# Autodesk Inventor assembly: Cup_Dispenser
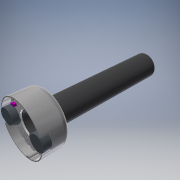
[picture p0: Inventor's stored thumbnail of the model, 180x180]
Saved by Autodesk Inventor 2016 (Build 200138000, 138)
## iProperties
Created: 2015-07-19
Part Number: Cup_Dispenser
Document SubType Name: Assembly
Designer: bastli
Author: bastli
## Documents named in this file (9)
- C:\Users\3DPrinterUser\Documents\GitHub\BarBot\Conception\Mechanical\Cup_Dispenser_3\Cup_Dispenser.iam
- C:\Users\3DPrinterUser\Documents\GitHub\BarBot\Conception\Mechanical\Cup_Dispenser_3\Fixture.ipt
- C:\Users\3DPrinterUser\Documents\GitHub\BarBot\Conception\Mechanical\Cup_Dispenser_3\Transmission.ipt
- C:\Users\3DPrinterUser\Documents\GitHub\BarBot\Conception\Mechanical\Cup_Dispenser\Cup_Dispenser_Pipe.ipt
- C:\Users\3DPrinterUser\Documents\GitHub\BarBot\Conception\Mechanical\Cup_Dispenser_3\Nema 11.ipt
- C:\Users\3DPrinterUser\Documents\GitHub\BarBot\Conception\Mechanical\Cup_Dispenser_3\Endstop_Fixture.ipt
- C:\Users\3DPrinterUser\Documents\GitHub\BarBot\Conception\Mechanical\Cup_Dispenser_3\Board_Shape.ipt
- C:\Users\3DPrinterUser\Documents\GitHub\BarBot\Conception\Mechanical\Cup_Dispenser_3\Board_Offset_Holder.ipt
- C:\Users\3DPrinterUser\Documents\GitHub\BarBot\Conception\Mechanical\Cup_Dispenser_3\Hull.ipt
## Components (17 placed, 8 different names)
1. Cup_Dispenser_Pipe:1 — Rotational:5
2. Fixture:1 — Rotational:5, Rigid:5, Rigid:6, Rigid:7, Rotational:8, Rotational:9, Rotational:10, Rotational:11, Rotational:12, Rotational:13, Flush:1, Rotational:14
3. Transmission:1 — Rotational:6
4. Nema 11:1 — Rigid:5, Rotational:6
5. Nema 11:2 — Rigid:6, Rotational:7
6. Transmission:2 — Rotational:7
7. Endstop_Fixture:1 — Rigid:7
8. Endstop_Fixture:2 — Rotational:8
9. Board_Shape:1 — Insert:2
10. Board_Offset_Holder:1 — Rotational:9, Insert:1
11. Board_Offset_Holder:2 — Rotational:10
12. Board_Offset_Holder:3 — Rotational:11
13. Board_Offset_Holder:4 — Rotational:12, Mate:1
14. Board_Offset_Holder:5 — Rotational:13
15. Hull:1 — Flush:1
16. Board_Shape:2 — Insert:1, Mate:1
17. Board_Offset_Holder:6 — Rotational:14, Insert:2
## Relationships (17: RevoluteJoint 10, WeldJoint 3, Insert 2, Flush 1, Mate 1)
- Rotational:5 [RevoluteJoint]: Cup_Dispenser_Pipe:1 ↔ Fixture:1
- Rigid:5 [WeldJoint]: Fixture:1 ↔ Nema 11:1
- Rigid:6 [WeldJoint]: Fixture:1 ↔ Nema 11:2
- Rotational:6 [RevoluteJoint]: Transmission:1 ↔ Nema 11:1
- Rotational:7 [RevoluteJoint]: Nema 11:2 ↔ Transmission:2
- Rigid:7 [WeldJoint]: Fixture:1 ↔ Endstop_Fixture:1
- Rotational:8 [RevoluteJoint]: Fixture:1 ↔ Endstop_Fixture:2
- Rotational:9 [RevoluteJoint]: Fixture:1 ↔ Board_Offset_Holder:1
- Rotational:10 [RevoluteJoint]: Fixture:1 ↔ Board_Offset_Holder:2
- Rotational:11 [RevoluteJoint]: Fixture:1 ↔ Board_Offset_Holder:3
- Rotational:12 [RevoluteJoint]: Fixture:1 ↔ Board_Offset_Holder:4
- Rotational:13 [RevoluteJoint]: Fixture:1 ↔ Board_Offset_Holder:5
- Flush:1: Fixture:1 ↔ Hull:1
- Insert:1: Board_Offset_Holder:1 ↔ Board_Shape:2
- Mate:1: Board_Offset_Holder:4 ↔ Board_Shape:2
- Rotational:14 [RevoluteJoint]: Fixture:1 ↔ Board_Offset_Holder:6
- Insert:2: Board_Shape:1 ↔ Board_Offset_Holder:6
